# Autodesk Inventor assembly: lift 1
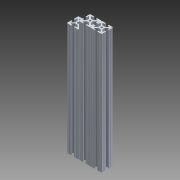
[picture p0: Inventor's stored thumbnail of the model, 180x180]
Saved by Autodesk Inventor 2015 (Build 190159000, 159)
## iProperties
Created: 2014-11-12
Part Number: lift 1
Document SubType Name: Assembly
Designer: kruegerma
Mass: 865.142 g
Surface Area: 3878.93 cm^2
Volume: 865.142 cm^3
Density: 1 g/cm^3
Author: kruegerma
## Documents named in this file (3)
- E:\lift 1.iam
- E:\8020 bottom piece.ipt
- E:\8020 middle piece.ipt
## Components (3 placed, 2 different names)
1. 8020 bottom piece:1 — Flush:1, Mate:1, Flush:5
2. 8020 middle piece:3 — Flush:2, Mate:2, Flush:6, Flush:7
3. 8020 middle piece:4 — Flush:1, Mate:1, Flush:2, Mate:2, Flush:5, Flush:6, Flush:7
## Relationships (7: Flush 5, Mate 2)
- Flush:1: 8020 bottom piece:1 ↔ 8020 middle piece:4
- Mate:1: 8020 bottom piece:1 ↔ 8020 middle piece:4
- Flush:2: 8020 middle piece:3 ↔ 8020 middle piece:4
- Mate:2: 8020 middle piece:3 ↔ 8020 middle piece:4
- Flush:5: 8020 bottom piece:1 ↔ 8020 middle piece:4
- Flush:6: 8020 middle piece:3 ↔ 8020 middle piece:4
- Flush:7: 8020 middle piece:3 ↔ 8020 middle piece:4
